# Autodesk Inventor assembly: montaz_gps_bt
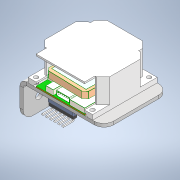
[picture p0: Inventor's stored thumbnail of the model, 180x180]
Saved by Autodesk Inventor 2020 (Build 240168000, 168)
## iProperties
Created: 2020-09-03
Part Number: montaz_gps_bt
Document SubType Name: Assembly
Designer: Hesekiel
Author: Hesekiel
## Documents named in this file (5)
- C:\Users\Hesekiel\Desktop\MUM\Mechanika\Mechanizm elewacji i elektronika Filip\CAD\montaz_gps_bt.iam
- C:\Users\Hesekiel\Desktop\MUM\Mechanika\Mechanizm elewacji i elektronika Filip\CAD\HC_05 Blue Tooth Module.ipt
- C:\Users\Hesekiel\Desktop\MUM\Mechanika\Mechanizm elewacji i elektronika Filip\CAD\plyta_montazowa_gps_bt.ipt
- C:\Users\Hesekiel\Desktop\MUM\Mechanika\Mechanizm elewacji i elektronika Filip\CAD\obudowa_gps_bt.ipt
- C:\Users\Hesekiel\Desktop\MUM\Mechanika\Mechanizm elewacji i elektronika Filip\CAD\Moduł GPS\EM406 GPS Module.ipt
## Components (4 placed, 4 different names)
1. HC_05 Blue Tooth Module:1 — Mate:5, Flush:2
2. plyta_montazowa_gps_bt:1 — Mate:1, Mate:2, Mate:3, Mate:4, Flush:1, Mate:5, Flush:2
3. obudowa_gps_bt:1 — Mate:1, Mate:2, Mate:3
4. EM406 GPS Module:1 — Mate:4, Flush:1
## Relationships (7: Mate 5, Flush 2)
- Mate:1: plyta_montazowa_gps_bt:1 ↔ obudowa_gps_bt:1
- Mate:2: plyta_montazowa_gps_bt:1 ↔ obudowa_gps_bt:1
- Mate:3: plyta_montazowa_gps_bt:1 ↔ obudowa_gps_bt:1
- Mate:4: plyta_montazowa_gps_bt:1 ↔ EM406 GPS Module:1
- Flush:1: plyta_montazowa_gps_bt:1 ↔ EM406 GPS Module:1
- Mate:5: HC_05 Blue Tooth Module:1 ↔ plyta_montazowa_gps_bt:1
- Flush:2: HC_05 Blue Tooth Module:1 ↔ plyta_montazowa_gps_bt:1
